# Autodesk Inventor assembly: R07-100-RNEA
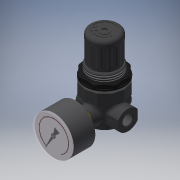
[picture p0: Inventor's stored thumbnail of the model, 180x180]
Saved by Autodesk Inventor 2016 (Build 200138000, 138)
## iProperties
Category: Pneumatics
Company: Autodesk Inc.
Created: 2015-12-11
Part Number: R07-100-RNEA
Document SubType Name: Assembly
Designer: Autodesk Inc.
Catalog Web Link: http://store.norgren.com/us/en/search.aspx?q=r07-100-rnea
Vendor: Norgren
Description: Main Regulator (assembled)
Author: Autodesk Inc.
## Documents named in this file (4)
- E:\Improved  2011 Robot\FRC KOP 2016\Pneumatics\Pneu_Norgren_R07-100-RNEA.iam
- E:\Improved  2011 Robot\FRC KOP 2016\Pneumatics\Parts\Pneumatics_Norgren_R07-100-RNEA.ipt
- E:\Improved  2011 Robot\FRC KOP 2016\Pneumatics\Parts\Pneumatics_Norgren_18-025-003_Panel Nut.ipt
- E:\Improved  2011 Robot\FRC KOP 2016\Pneumatics\Pneu_Norgren_18-013-212.iam
## Components (3 placed, 3 different names)
1. Pneumatics_Norgren_R07-100-RNEA:1 — Mate:3, Insert:1
2. Pneumatics_Norgren_18-025-003_Panel Nut:1 — Mate:3
3. Pneu_Norgren_18-013-212:1 [sub-assembly] — Insert:1
## Relationships (2: Mate 1, Insert 1)
- Mate:3: Pneumatics_Norgren_R07-100-RNEA:1 ↔ Pneumatics_Norgren_18-025-003_Panel Nut:1
- Insert:1: Pneumatics_Norgren_R07-100-RNEA:1 ↔ Pneu_Norgren_18-013-212:1
